# Autodesk Inventor assembly: Train asembley
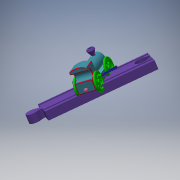
[picture p0: Inventor's stored thumbnail of the model, 180x180]
Saved by Autodesk Inventor 2017.1 (Build 211199000, 199)
## iProperties
Created: 2017-04-26
Part Number: Train asembley
Document SubType Name: Assembly
Designer: 196918
Author: 196918
## Documents named in this file (11)
- C:\Users\196918\Desktop\Train asembley.iam
- C:\Users\196918\Desktop\Cow pusher.ipt
- C:\Users\196918\Desktop\Train locomotive.ipt
- C:\Users\196918\Desktop\Train smoke stack.ipt
- C:\Users\196918\Desktop\Screw (train).ipt
- C:\Users\196918\Desktop\Washer (Train).ipt
- C:\Users\196918\Desktop\hex nut.ipt
- C:\Users\196918\Desktop\linkage arm.ipt
- C:\Users\196918\Desktop\linkage peg.ipt
- C:\Users\196918\Desktop\train track.ipt
- C:\Users\196918\Desktop\train wheel..ipt
## Components (20 placed, 10 different names)
1. Cow pusher:1 — Mate:1, Mate:2
2. Train locomotive:1 — Rigid:1, Mate:1, Mate:2, Rotational:1, Rotational:3, Rotational:4, Rotational:9, Rotational:10, Rotational:15
3. Train smoke stack:1 — Rigid:1
4. Screw (train):1 — Rotational:2
5. Washer (Train):1 — Rotational:1, Rotational:2
6. hex nut:1 — Rotational:7
7. linkage arm:1 — Mate:3, Mate:4, Mate:5, Mate:6
8. linkage peg:1 — Rotational:6
9. linkage arm:2 — Rotational:14, Mate:9, Cylindrical:1, Rotational:16
10. train track:1 — Rotational:15
11. train wheel.:1 — Rotational:3, Mate:3, Mate:6, Rotational:5, Rotational:8
12. train wheel.:2 — Rotational:4, Mate:4, Mate:5, Rotational:6, Rotational:7
13. train wheel.:3 — Rotational:9, Rotational:12, Cylindrical:1
14. train wheel.:4 — Rotational:10, Rotational:11, Mate:8
15. linkage peg:2 — Rotational:5
16. hex nut:2 — Rotational:8
17. hex nut:3 — Rotational:11
18. hex nut:4 — Rotational:12
19. linkage peg:3 — Mate:9, Rotational:16
20. linkage peg:4 — Rotational:14, Mate:8
## Relationships (25: RevoluteJoint 15, Mate 8, WeldJoint 1, CylindricalJoint 1)
- Rigid:1 [WeldJoint]: Train locomotive:1 ↔ Train smoke stack:1
- Mate:1: Cow pusher:1 ↔ Train locomotive:1
- Mate:2: Cow pusher:1 ↔ Train locomotive:1
- Rotational:1 [RevoluteJoint]: Train locomotive:1 ↔ Washer (Train):1
- Rotational:2 [RevoluteJoint]: Screw (train):1 ↔ Washer (Train):1
- Rotational:3 [RevoluteJoint]: Train locomotive:1 ↔ train wheel.:1
- Rotational:4 [RevoluteJoint]: Train locomotive:1 ↔ train wheel.:2
- Mate:3: linkage arm:1 ↔ train wheel.:1
- Mate:4: linkage arm:1 ↔ train wheel.:2
- Mate:5: linkage arm:1 ↔ train wheel.:2
- Mate:6: linkage arm:1 ↔ train wheel.:1
- Rotational:5 [RevoluteJoint]: train wheel.:1 ↔ linkage peg:2
- Rotational:6 [RevoluteJoint]: linkage peg:1 ↔ train wheel.:2
- Rotational:7 [RevoluteJoint]: hex nut:1 ↔ train wheel.:2
- Rotational:8 [RevoluteJoint]: train wheel.:1 ↔ hex nut:2
- Rotational:9 [RevoluteJoint]: Train locomotive:1 ↔ train wheel.:3
- Rotational:10 [RevoluteJoint]: Train locomotive:1 ↔ train wheel.:4
- Rotational:11 [RevoluteJoint]: train wheel.:4 ↔ hex nut:3
- Rotational:12 [RevoluteJoint]: train wheel.:3 ↔ hex nut:4
- Rotational:14 [RevoluteJoint]: linkage arm:2 ↔ linkage peg:4
- Rotational:15 [RevoluteJoint]: Train locomotive:1 ↔ train track:1
- Mate:8: train wheel.:4 ↔ linkage peg:4
- Mate:9: linkage arm:2 ↔ linkage peg:3
- Cylindrical:1: linkage arm:2 ↔ train wheel.:3
- Rotational:16 [RevoluteJoint]: linkage arm:2 ↔ linkage peg:3
